# Autodesk Inventor assembly: тело фулл
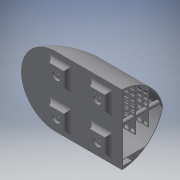
[picture p0: Inventor's stored thumbnail of the model, 180x180]
Saved by Autodesk Inventor 2019 (Build 230136000, 136)
## iProperties
Created: 2019-09-06
Part Number: тело фулл
Material: Типовые
Document SubType Name: Assembly
Designer: Iliga
Author: Iliga
## Documents named in this file (3)
- C:\Users\Iliga\Desktop\робот\тело фулл.iam
- C:\Users\Iliga\Desktop\робот\тело.ipt
- C:\Users\Iliga\Desktop\робот\правое надкрылье.ipt
## Components (2 placed, 2 different names)
1. тело основа:1 — Заподлицо:3, Совмещение:2, Совмещение:3
2. правое надкрылье:1 — Заподлицо:3, Совмещение:2, Совмещение:3
## Relationships (3: Mate 2, Flush 1)
- Заподлицо:3 [Flush]: тело основа:1 ↔ правое надкрылье:1
- Совмещение:2 [Mate]: тело основа:1 ↔ правое надкрылье:1
- Совмещение:3 [Mate]: тело основа:1 ↔ правое надкрылье:1
